# Autodesk Inventor assembly: 39092
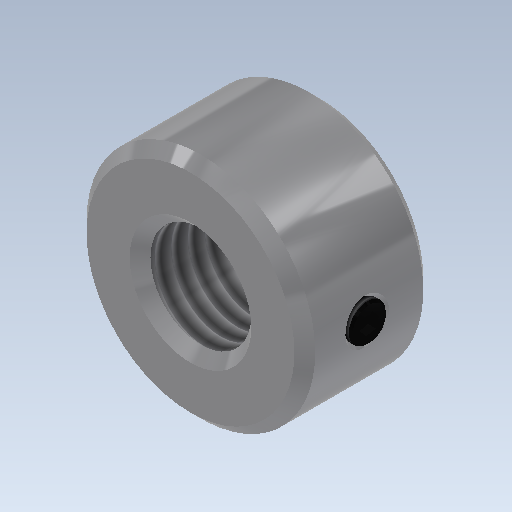
[picture p0: Inventor's stored thumbnail of the model, 512x512]
Saved by Autodesk Inventor 2020.1 (Build 241239000, 239)
## iProperties
Created: 2017-01-02
Part Number: 39092
Document SubType Name: Assembly
Designer: Autodesk Inc.
Catalog Web Link: http://www.tetrixrobotics.com/TETRIX_Axle_Set_Collars
Vendor: Tetrix
Category: Collars
Company: Autodesk Inc.
Author: Autodesk Inc.
## Documents named in this file (3)
- B:\Documents\GitHub\AO_Robotics\CAD\Parts Kits\FTC Tetrix KOP Organized (7-24-19)\Axle Hardware\Tetrix_39092.iam
- B:\Documents\GitHub\AO_Robotics\CAD\Parts Kits\FTC Tetrix KOP Organized (7-24-19)\Axle Hardware\Assembly Components\Tetrix_39092_Collar.ipt
- B:\Documents\GitHub\AO_Robotics\CAD\Parts Kits\FTC Tetrix KOP Organized (7-24-19)\Axle Hardware\Assembly Components\Tetrix_39092_Screw.ipt
## Components (2 placed, 2 different names)
1. Tetrix_39092_Collar — Mate:1
2. Tetrix_39092_Screw — Mate:1
## Relationships (1: Mate 1)
- Mate:1: Tetrix_39092_Collar ↔ Tetrix_39092_Screw
